# Autodesk Inventor assembly: Mao-robotica-alpha
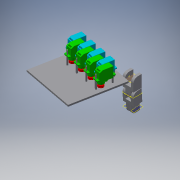
[picture p0: Inventor's stored thumbnail of the model, 180x180]
Saved by Autodesk Inventor 2018 (Build 220112000, 112)
## iProperties
Created: 2017-06-01
Part Number: Mao-robotica-alpha
Material: Genérico
Document SubType Name: Assembly
Designer: Vitor
Author: Vitor
## Documents named in this file (7)
- C:\Users\Vitor\Documents\Autodesk\Mao-Robotica\Mao-robotica-alpha.iam
- C:\Users\Vitor\Documents\Autodesk\Mao-Robotica\Palma.ipt
- C:\Users\Vitor\Documents\Autodesk\Mao-Robotica\Motor.ipt
- C:\Users\Vitor\Documents\Autodesk\Mao-Robotica\Polia.ipt
- C:\Users\Vitor\Documents\Autodesk\Mao-Robotica\Falange-proximal.ipt
- C:\Users\Vitor\Documents\Autodesk\Mao-Robotica\Falange-media.ipt
- C:\Users\Vitor\Documents\Autodesk\Mao-Robotica\Falange-media2.ipt
## Components (20 placed, 6 different names)
1. Palma:1 — Inserir:26, Inserir:27, Inserir:28, Inserir:29, Inserir:30, Inserir:31, Inserir:32, Inserir:33, Inserir:34, Inserir:35, Inserir:36, Inserir:37, Inserir:38, Inserir:39, Inserir:40, Inserir:41
2. Motor:1 — Inserir:7, Inserir:30, Inserir:31
3. Motor:2 — Inserir:1, Inserir:26, Inserir:27
4. Motor:3 — Inserir:8, Inserir:32, Inserir:33
5. Motor:4 — Inserir:9, Inserir:34, Inserir:35
6. Motor:5 — Inserir:10, Inserir:36, Inserir:37
7. Motor:6 — Inserir:11, Inserir:38, Inserir:39
8. Motor:7 — Inserir:12, Inserir:40, Inserir:41
9. Motor:8 — Inserir:4, Inserir:28, Inserir:29
10. Polia:1 — Inserir:4
11. Polia:2 — Inserir:12
12. Polia:3 — Inserir:11
13. Polia:4 — Inserir:10
14. Polia:5 — Inserir:9
15. Polia:6 — Inserir:8
16. Polia:7 — Inserir:7
17. Polia:8 — Inserir:1
18. Falange-proximal:1 — Inserir:25
19. Falange-media:1
20. Falange-media2:1 — Inserir:25
## Relationships (25: Insert 25)
- Inserir:1: Motor:2 ↔ Polia:8
- Inserir:4: Motor:8 ↔ Polia:1
- Inserir:7: Motor:1 ↔ Polia:7
- Inserir:8: Motor:3 ↔ Polia:6
- Inserir:9: Motor:4 ↔ Polia:5
- Inserir:10: Motor:5 ↔ Polia:4
- Inserir:11: Motor:6 ↔ Polia:3
- Inserir:12: Motor:7 ↔ Polia:2
- Inserir:25 (0.5 mm): Falange-proximal:1 ↔ Falange-media2:1
- Inserir:26: Palma:1 ↔ Motor:2
- Inserir:27: Palma:1 ↔ Motor:2
- Inserir:28: Palma:1 ↔ Motor:8
- Inserir:29: Palma:1 ↔ Motor:8
- Inserir:30: Palma:1 ↔ Motor:1
- Inserir:31: Palma:1 ↔ Motor:1
- Inserir:32: Palma:1 ↔ Motor:3
- Inserir:33: Palma:1 ↔ Motor:3
- Inserir:34: Palma:1 ↔ Motor:4
- Inserir:35: Palma:1 ↔ Motor:4
- Inserir:36: Palma:1 ↔ Motor:5
- Inserir:37: Palma:1 ↔ Motor:5
- Inserir:38: Palma:1 ↔ Motor:6
- Inserir:39: Palma:1 ↔ Motor:6
- Inserir:40: Palma:1 ↔ Motor:7
- Inserir:41: Palma:1 ↔ Motor:7
